# Autodesk Inventor assembly: PC104 STACK USB INTERFACE
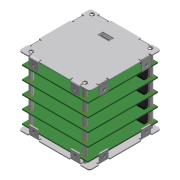
[picture p0: Inventor's stored thumbnail of the model, 180x180]
Saved by Autodesk Inventor 2018 (Build 220112000, 112)
## iProperties
Created: 2018-12-12
Part Number: PC104 STACK USB INTERFACE
Document SubType Name: Assembly
Designer: R.P.SMITH
Mass: 230.284 g
Surface Area: 2018.76 cm^2
Volume: 144.259 cm^3
Density: 1.59633 g/cm^3
Author: R.P.SMITH
## Documents named in this file (11)
- D:\Documents\College\Semesters\4 - Fall\Senior Project 2\CADD Files\PC104 STACK USB INTERFACE.iam
- D:\Documents\College\Semesters\4 - Fall\Senior Project 2\CADD Files\PC104 ISA BOARD.iam
- D:\Documents\College\Semesters\4 - Fall\Senior Project 2\CADD Files\McMaster\93505A925_ALUM MALE-FEM THRDED HEX STANDOFF.ipt
- D:\Documents\College\Semesters\4 - Fall\Senior Project 2\CADD Files\PC104 ISA MODIFIED END.iam
- D:\Documents\College\Semesters\4 - Fall\Senior Project 2\CADD Files\McMaster\91780A534_ALUM FEM THRDED HEX STANDOFF.ipt
- D:\Documents\College\Semesters\4 - Fall\Senior Project 2\CADD Files\McMaster\92510A692_ALUM UNTHRD SPACER.ipt
- D:\Documents\College\Semesters\4 - Fall\Senior Project 2\CADD Files\McMaster\91772A106_18-8 SS PAN HEAD PHILLIPS MACHINE SCREW.ipt
- D:\Documents\College\Semesters\4 - Fall\Senior Project 2\CADD Files\Custom Parts\END MOUNT PC104 BOTTOM.iam
- D:\Documents\College\Semesters\4 - Fall\Senior Project 2\CADD Files\McMaster\91772A112_18-8 SS PAN HEAD PHILLIPS MACHINE SCREW.ipt
- D:\Documents\College\Semesters\4 - Fall\Senior Project 2\CADD Files\Mouser\614004135023.ipt
- D:\Documents\College\Semesters\4 - Fall\Senior Project 2\CADD Files\Custom Parts\END MOUNT PC104 TOP USB.iam
## Components (40 placed, 10 different names)
1. PC104 ISA MODIFIED END:1 [sub-assembly] — Mate:13, Mate:14, Mate:15, Insert:25, Insert:26, Insert:27, Insert:28
2. 91780A534_ALUM FEM THRDED HEX STANDOFF:1 — Insert:21
3. 91780A534_ALUM FEM THRDED HEX STANDOFF:2 — Insert:24
4. 91780A534_ALUM FEM THRDED HEX STANDOFF:3 — Insert:23
5. 91780A534_ALUM FEM THRDED HEX STANDOFF:4 — Insert:22
6. PC104 ISA BOARD:2 [sub-assembly] — Mate:4, Mate:5, Mate:6, Insert:1, Insert:4, Insert:6, Insert:8, Mate:13, Mate:14, Mate:15, Insert:21, Insert:22, Insert:23, Insert:24
7. 93505A925_ALUM MALE-FEM THRDED HEX STANDOFF:1 — Insert:1
8. 93505A925_ALUM MALE-FEM THRDED HEX STANDOFF:4 — Insert:4
9. 93505A925_ALUM MALE-FEM THRDED HEX STANDOFF:6 — Insert:6
10. 93505A925_ALUM MALE-FEM THRDED HEX STANDOFF:8 — Insert:8
11. PC104 ISA BOARD:3 [sub-assembly] — Mate:4, Mate:5, Mate:6, Insert:9, Insert:10, Insert:11, Insert:12, Mate:7, Mate:8, Mate:9
12. 93505A925_ALUM MALE-FEM THRDED HEX STANDOFF:9 — Insert:12
13. 93505A925_ALUM MALE-FEM THRDED HEX STANDOFF:10 — Insert:10
14. 93505A925_ALUM MALE-FEM THRDED HEX STANDOFF:11 — Insert:11
15. 93505A925_ALUM MALE-FEM THRDED HEX STANDOFF:12 — Insert:9
16. PC104 ISA BOARD:4 [sub-assembly] — Mate:7, Mate:8, Mate:9, Insert:13, Insert:14, Insert:15, Insert:16, Mate:10, Mate:11, Mate:12
17. 93505A925_ALUM MALE-FEM THRDED HEX STANDOFF:13 — Insert:16
18. 93505A925_ALUM MALE-FEM THRDED HEX STANDOFF:14 — Insert:13
19. 93505A925_ALUM MALE-FEM THRDED HEX STANDOFF:15 — Insert:14
20. 93505A925_ALUM MALE-FEM THRDED HEX STANDOFF:16 — Insert:15
21. PC104 ISA BOARD:5 [sub-assembly] — Mate:10, Mate:11, Mate:12, Insert:17, Insert:18, Insert:19, Insert:20, Mate:16, Mate:17, Flush:1
22. 93505A925_ALUM MALE-FEM THRDED HEX STANDOFF:17 — Insert:20
23. 93505A925_ALUM MALE-FEM THRDED HEX STANDOFF:18 — Insert:19, Flush:2, Mate:18
24. 93505A925_ALUM MALE-FEM THRDED HEX STANDOFF:19 — Insert:18
25. 93505A925_ALUM MALE-FEM THRDED HEX STANDOFF:20 — Insert:17, Mate:19
26. 92510A692_ALUM UNTHRD SPACER:1 — Insert:25, Insert:35
27. 92510A692_ALUM UNTHRD SPACER:2 — Insert:28
28. 92510A692_ALUM UNTHRD SPACER:3 — Insert:26, Insert:36
29. 92510A692_ALUM UNTHRD SPACER:4 — Insert:27
30. END MOUNT PC104 TOP USB:1 [sub-assembly] — Flush:2, Mate:18, Mate:19, Insert:41, Insert:42, Insert:43, Insert:44
31. 91772A106_18-8 SS PAN HEAD PHILLIPS MACHINE SCREW:1 — Insert:44
32. 91772A106_18-8 SS PAN HEAD PHILLIPS MACHINE SCREW:2 — Insert:43
33. 91772A106_18-8 SS PAN HEAD PHILLIPS MACHINE SCREW:3 — Insert:42
34. 91772A106_18-8 SS PAN HEAD PHILLIPS MACHINE SCREW:4 — Insert:41
35. END MOUNT PC104 BOTTOM:1 [sub-assembly] — Insert:35, Insert:36, Insert:37, Insert:38, Insert:39, Insert:40
36. 91772A112_18-8 SS PAN HEAD PHILLIPS MACHINE SCREW:1 — Insert:37
37. 91772A112_18-8 SS PAN HEAD PHILLIPS MACHINE SCREW:2 — Insert:38
38. 91772A112_18-8 SS PAN HEAD PHILLIPS MACHINE SCREW:3 — Insert:39
39. 91772A112_18-8 SS PAN HEAD PHILLIPS MACHINE SCREW:4 — Insert:40
40. 614004135023:1 — Mate:16, Mate:17, Flush:1
## Relationships (52: Insert 34, Mate 16, Flush 2)
- Mate:4 (15.875 mm): PC104 ISA BOARD:2 ↔ PC104 ISA BOARD:3
- Mate:5: PC104 ISA BOARD:2 ↔ PC104 ISA BOARD:3
- Mate:6: PC104 ISA BOARD:2 ↔ PC104 ISA BOARD:3
- Insert:1: PC104 ISA BOARD:2 ↔ 93505A925_ALUM MALE-FEM THRDED HEX STANDOFF:1
- Insert:4: PC104 ISA BOARD:2 ↔ 93505A925_ALUM MALE-FEM THRDED HEX STANDOFF:4
- Insert:6: PC104 ISA BOARD:2 ↔ 93505A925_ALUM MALE-FEM THRDED HEX STANDOFF:6
- Insert:8: PC104 ISA BOARD:2 ↔ 93505A925_ALUM MALE-FEM THRDED HEX STANDOFF:8
- Insert:9: PC104 ISA BOARD:3 ↔ 93505A925_ALUM MALE-FEM THRDED HEX STANDOFF:12
- Insert:10: PC104 ISA BOARD:3 ↔ 93505A925_ALUM MALE-FEM THRDED HEX STANDOFF:10
- Insert:11: PC104 ISA BOARD:3 ↔ 93505A925_ALUM MALE-FEM THRDED HEX STANDOFF:11
- Insert:12: PC104 ISA BOARD:3 ↔ 93505A925_ALUM MALE-FEM THRDED HEX STANDOFF:9
- Mate:7: PC104 ISA BOARD:3 ↔ PC104 ISA BOARD:4
- Mate:8: PC104 ISA BOARD:3 ↔ PC104 ISA BOARD:4
- Mate:9 (15.875 mm): PC104 ISA BOARD:3 ↔ PC104 ISA BOARD:4
- Insert:13: PC104 ISA BOARD:4 ↔ 93505A925_ALUM MALE-FEM THRDED HEX STANDOFF:14
- Insert:14: PC104 ISA BOARD:4 ↔ 93505A925_ALUM MALE-FEM THRDED HEX STANDOFF:15
- Insert:15: PC104 ISA BOARD:4 ↔ 93505A925_ALUM MALE-FEM THRDED HEX STANDOFF:16
- Insert:16: PC104 ISA BOARD:4 ↔ 93505A925_ALUM MALE-FEM THRDED HEX STANDOFF:13
- Mate:10 (15.875 mm): PC104 ISA BOARD:4 ↔ PC104 ISA BOARD:5
- Mate:11: PC104 ISA BOARD:4 ↔ PC104 ISA BOARD:5
- Mate:12: PC104 ISA BOARD:4 ↔ PC104 ISA BOARD:5
- Insert:17: PC104 ISA BOARD:5 ↔ 93505A925_ALUM MALE-FEM THRDED HEX STANDOFF:20
- Insert:18: PC104 ISA BOARD:5 ↔ 93505A925_ALUM MALE-FEM THRDED HEX STANDOFF:19
- Insert:19: PC104 ISA BOARD:5 ↔ 93505A925_ALUM MALE-FEM THRDED HEX STANDOFF:18
- Insert:20: PC104 ISA BOARD:5 ↔ 93505A925_ALUM MALE-FEM THRDED HEX STANDOFF:17
- Mate:13 (15.875 mm): PC104 ISA MODIFIED END:1 ↔ PC104 ISA BOARD:2
- Mate:14: PC104 ISA MODIFIED END:1 ↔ PC104 ISA BOARD:2
- Mate:15: PC104 ISA MODIFIED END:1 ↔ PC104 ISA BOARD:2
- Insert:21: 91780A534_ALUM FEM THRDED HEX STANDOFF:1 ↔ PC104 ISA BOARD:2
- Insert:22: 91780A534_ALUM FEM THRDED HEX STANDOFF:4 ↔ PC104 ISA BOARD:2
- Insert:23: 91780A534_ALUM FEM THRDED HEX STANDOFF:3 ↔ PC104 ISA BOARD:2
- Insert:24: 91780A534_ALUM FEM THRDED HEX STANDOFF:2 ↔ PC104 ISA BOARD:2
- Insert:25: PC104 ISA MODIFIED END:1 ↔ 92510A692_ALUM UNTHRD SPACER:1
- Insert:26: PC104 ISA MODIFIED END:1 ↔ 92510A692_ALUM UNTHRD SPACER:3
- Insert:27: PC104 ISA MODIFIED END:1 ↔ 92510A692_ALUM UNTHRD SPACER:4
- Insert:28: PC104 ISA MODIFIED END:1 ↔ 92510A692_ALUM UNTHRD SPACER:2
- Insert:35: 92510A692_ALUM UNTHRD SPACER:1 ↔ END MOUNT PC104 BOTTOM:1
- Insert:36: 92510A692_ALUM UNTHRD SPACER:3 ↔ END MOUNT PC104 BOTTOM:1
- Insert:37: END MOUNT PC104 BOTTOM:1 ↔ 91772A112_18-8 SS PAN HEAD PHILLIPS MACHINE SCREW:1
- Insert:38: END MOUNT PC104 BOTTOM:1 ↔ 91772A112_18-8 SS PAN HEAD PHILLIPS MACHINE SCREW:2
- Insert:39: END MOUNT PC104 BOTTOM:1 ↔ 91772A112_18-8 SS PAN HEAD PHILLIPS MACHINE SCREW:3
- Insert:40: END MOUNT PC104 BOTTOM:1 ↔ 91772A112_18-8 SS PAN HEAD PHILLIPS MACHINE SCREW:4
- Mate:16: PC104 ISA BOARD:5 ↔ 614004135023:1
- Mate:17 (5 mm): PC104 ISA BOARD:5 ↔ 614004135023:1
- Flush:1 (30 mm): PC104 ISA BOARD:5 ↔ 614004135023:1
- Flush:2: 93505A925_ALUM MALE-FEM THRDED HEX STANDOFF:18 ↔ END MOUNT PC104 TOP USB:1
- Mate:18: 93505A925_ALUM MALE-FEM THRDED HEX STANDOFF:18 ↔ END MOUNT PC104 TOP USB:1
- Mate:19: 93505A925_ALUM MALE-FEM THRDED HEX STANDOFF:20 ↔ END MOUNT PC104 TOP USB:1
- Insert:41: END MOUNT PC104 TOP USB:1 ↔ 91772A106_18-8 SS PAN HEAD PHILLIPS MACHINE SCREW:4
- Insert:42: END MOUNT PC104 TOP USB:1 ↔ 91772A106_18-8 SS PAN HEAD PHILLIPS MACHINE SCREW:3
- Insert:43: END MOUNT PC104 TOP USB:1 ↔ 91772A106_18-8 SS PAN HEAD PHILLIPS MACHINE SCREW:2
- Insert:44: END MOUNT PC104 TOP USB:1 ↔ 91772A106_18-8 SS PAN HEAD PHILLIPS MACHINE SCREW:1
